# Autodesk Inventor assembly: 2v2 LWL Robot
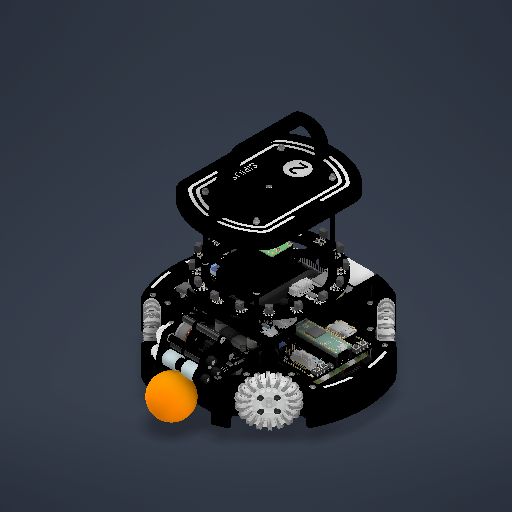
[picture p0: Inventor's stored thumbnail of the model, 512x512]
Saved by Autodesk Inventor 2026.1 (Build 301233020, 233B)
## iProperties
Created: 2026-04-03
Part Number: 2v2 LWL Robot
Document SubType Name: Assembly
Designer: Bahaa
Mass: 1441.25 g
Surface Area: 8202.25 cm^2
Volume: 790.623 cm^3
Density: 1.82292 g/cm^3
Author: Bahaa
## Documents named in this file (23)
- C:\Users\Bahaa\Nextcloud2\CAD\25-26\V2\2v2 LWL Robot.iam
- C:\Users\Bahaa\Nextcloud2\CAD\25-26\V2\Bottom Ring.ipt
- C:\Users\Bahaa\Nextcloud2\CAD\25-26\V2\Motor Assembly.iam
- C:\Users\Bahaa\Nextcloud2\CAD\25-26\V2\Top Ring.ipt
- C:\Users\Bahaa\Nextcloud2\CAD\25-26\V2\Side Wall.ipt
- C:\Users\Bahaa\Nextcloud2\CAD\25-26\V2\Battery Cover.ipt
- C:\Users\Bahaa\Nextcloud2\CAD\25-26\V2\Parts\SLS Quantum 1300mAh 4S1P 14,8V 65C.ipt
- C:\Users\Bahaa\Nextcloud2\CAD\25-26\V2\Solenoid JF-0826B\Solenoid JF-0826B\Solenoid.iam
- C:\Users\Bahaa\Nextcloud2\CAD\25-26\V2\Central Assembly.iam
- C:\Users\Bahaa\Nextcloud2\CAD\25-26\V2\Dribbler\Dribbler V2\Dribbler.iam
- C:\Users\Bahaa\Nextcloud2\CAD\25-26\V2\Ball.ipt
- C:\Users\Bahaa\Documents\Inventor\Content Center Files\R2026\en-US\DIN 7991(2)\DIN 7991 - M3x8.ipt
- C:\Users\Bahaa\Documents\Inventor\Content Center Files\R2026\en-US\DIN 912\DIN 912 - M3 x 0,5 x 5 x 3,75.ipt
- C:\Users\Bahaa\Nextcloud2\CAD\25-26\V2\Boards\Lineboard\Lineboard\Lineboard.iam
- C:\Users\Bahaa\Nextcloud2\CAD\25-26\V2\Boards\Logic Board\Logic Board\Logic Board.iam
- C:\Users\Bahaa\Nextcloud2\CAD\25-26\V2\Boards\Motor Board R\Motor Board R\Motor Board R.iam
- C:\Users\Bahaa\Nextcloud2\CAD\25-26\V2\Boards\Motor Board L\Motor Board L\Motor Board L.iam
- C:\Users\Bahaa\Nextcloud2\CAD\25-26\V2\Boards\Power Board\Power Board\Power Board.iam
- C:\Users\Bahaa\Documents\Inventor\Content Center Files\R2026\en-US\DIN 934\DIN 934 - M3 x 0,5.ipt
- C:\Users\Bahaa\Nextcloud2\CAD\25-26\V2\Boards\Kicker Board\Kicker Board\Kicker Board.iam
- C:\Users\Bahaa\Nextcloud2\CAD\25-26\V2\Parts\LED.ipt
- C:\Users\Bahaa\Nextcloud2\CAD\25-26\V2\Parts\WP3DP3BT.ipt
- C:\Users\Bahaa\Nextcloud2\CAD\25-26\V2\Parts\XL6019 Joy-IT\XL6019 Joy-IT\XL6019 Joy-IT\XL6019 Joy-IT.iam
## Components (44 placed, 22 different names)
1. Central Assembly:1 [sub-assembly] — Mate:53, Mate:54, Mate:55, Insert:1, Insert:2, Insert:3, Insert:4, Insert:5, Insert:6, Insert:7, Insert:8
2. Dribbler:1 [sub-assembly] — Mate:56, Mate:57, Mate:58, Tangent:1, Mate:62, Mate:63
3. Ball:1 — Mate:59, Mate:60, Mate:61
4. Motor Board R:1 [sub-assembly] — Mate:73, Mate:74, Mate:75, Mate:80, Flush:59, Flush:60
5. Motor Board L:1 [sub-assembly] — Mate:76, Mate:77, Mate:78, Mate:79, Flush:57, Flush:58
6. Power Board:1 [sub-assembly] — Mate:80, Flush:59, Flush:60
7. Kicker Board:1 [sub-assembly] — Mate:88, Mate:89, Mate:90, Insert:16, Insert:17
8. LED:1 — Mate:91, Mate:92
9. WP3DP3BT:1 — Mate:93, Mate:94
10. XL6019 Joy-IT:1 [sub-assembly] — Mate:95, Mate:97, Mate:98, Mate:99, Mate:100, Insert:18, Insert:19
11. DIN 934 - replaced by DIN EN 24032/28673/28674 M3:1 — Angle:3, Mate:97
12. DIN 934 - replaced by DIN EN 24032/28673/28674 M3:2 — Mate:96, Angle:4, Mate:98
13. DIN 912 - replaced by DIN EN ISO 4762 M3 x 5:18 — Insert:18
14. DIN 912 - replaced by DIN EN ISO 4762 M3 x 5:19 — Insert:19
15. Bottom Ring:1 — Mate:1, Mate:17, Mate:18, Flush:1, Mate:22, Mate:24, Mate:27, Mate:28, Mate:29, Mate:33, Mate:60, Angle:2, Mate:70, Mate:71, Mate:72, Mate:91, Mate:92, Mate:93, Mate:94
16. Top Ring:1 — Mate:4, Mate:23, Mate:25, Mate:26, Mate:30, Mate:48, Mate:53, Mate:54, Mate:55, Mate:56, Mate:57, Mate:58, Insert:9, Insert:10, Insert:11, Insert:12, Insert:13, Mate:88, Mate:89, Mate:90, Mate:95, Angle:3, Angle:4, Mate:99, Mate:100
17. Lineboard:1 [sub-assembly] — Mate:70, Mate:71, Mate:72
18. Logic Board:1 [sub-assembly] — Mate:79, Flush:57, Flush:58
19. Side Wall:1 — Flush:1, Mate:25, Mate:26, Mate:76, Mate:77, Mate:78
20. Side Wall:2 — Mate:22, Mate:23, Mate:24, Mate:73, Mate:74, Mate:75
21. Battery Cover:1 — Mate:27, Mate:28, Mate:29, Mate:30, Mate:32
22. SLS Quantum 1300mAh 4S1P 14,8V 65C:1 — Mate:32, Mate:33
23. Solenoid:1 [sub-assembly] — Mate:48
24. DIN 912 - replaced by DIN EN ISO 4762 M3 x 5:16 — Insert:16
25. DIN 912 - replaced by DIN EN ISO 4762 M3 x 5:17 — Insert:17
26. DIN 7991 M3x8:1 — Mate:62
27. DIN 7991 M3x8:2 — Mate:63
28. DIN 912 - replaced by DIN EN ISO 4762 M3 x 5:1 — Insert:1
29. DIN 912 - replaced by DIN EN ISO 4762 M3 x 5:2 — Insert:2
30. DIN 912 - replaced by DIN EN ISO 4762 M3 x 5:3 — Insert:3
31. DIN 912 - replaced by DIN EN ISO 4762 M3 x 5:4 — Insert:4
32. DIN 912 - replaced by DIN EN ISO 4762 M3 x 5:5 — Insert:5
33. DIN 912 - replaced by DIN EN ISO 4762 M3 x 5:6 — Insert:6
34. DIN 912 - replaced by DIN EN ISO 4762 M3 x 5:7 — Insert:7
35. DIN 912 - replaced by DIN EN ISO 4762 M3 x 5:8 — Insert:8
36. DIN 912 - replaced by DIN EN ISO 4762 M3 x 5:9 — Insert:9
37. DIN 912 - replaced by DIN EN ISO 4762 M3 x 5:10 — Insert:10
38. DIN 912 - replaced by DIN EN ISO 4762 M3 x 5:11 — Insert:11
39. DIN 912 - replaced by DIN EN ISO 4762 M3 x 5:12 — Insert:12
40. DIN 912 - replaced by DIN EN ISO 4762 M3 x 5:13 — Insert:13
41. Motor Assembly:1 [sub-assembly] — Mate:1, Mate:17, Mate:18
42. Motor Assembly:2 [sub-assembly] — Mate:4
43. Motor Assembly:3 [sub-assembly]
44. Motor Assembly:4 [sub-assembly]
## Component patterns: Motor Assemblies (4 elements)
## Relationships (78: Mate 51, Insert 17, Flush 6, Angle 3, Tangent 1)
- Mate:1: Bottom Ring:1 ↔ Motor Assembly:1
- Mate:4: Top Ring:1 ↔ Motor Assembly:2
- Mate:17: Bottom Ring:1 ↔ Motor Assembly:1
- Mate:18: Bottom Ring:1 ↔ Motor Assembly:1
- Flush:1: Bottom Ring:1 ↔ Side Wall:1
- Mate:22: Bottom Ring:1 ↔ Side Wall:2
- Mate:23: Top Ring:1 ↔ Side Wall:2
- Mate:24: Bottom Ring:1 ↔ Side Wall:2
- Mate:25: Top Ring:1 ↔ Side Wall:1
- Mate:26: Top Ring:1 ↔ Side Wall:1
- Mate:27: Bottom Ring:1 ↔ Battery Cover:1
- Mate:28: Bottom Ring:1 ↔ Battery Cover:1
- Mate:29: Bottom Ring:1 ↔ Battery Cover:1
- Mate:30: Top Ring:1 ↔ Battery Cover:1
- Mate:32 (0.25 mm): Battery Cover:1 ↔ SLS Quantum 1300mAh 4S1P 14,8V 65C:1
- Mate:33 (0.25 mm): Bottom Ring:1 ↔ SLS Quantum 1300mAh 4S1P 14,8V 65C:1
- Mate:48: Top Ring:1 ↔ Solenoid:1
- Mate:53: Central Assembly:1 ↔ Top Ring:1
- Mate:54: Central Assembly:1 ↔ Top Ring:1
- Mate:55: Central Assembly:1 ↔ Top Ring:1
- Mate:56: Dribbler:1 ↔ Top Ring:1
- Mate:57: Dribbler:1 ↔ Top Ring:1
- Mate:58: Dribbler:1 ↔ Top Ring:1
- Flush:56 (-11 mm)
- Mate:59 (21 mm): Ball:1
- Mate:60 (21 mm): Ball:1 ↔ Bottom Ring:1
- Mate:61: Ball:1
- Angle:2 (0 deg): Bottom Ring:1
- Tangent:1: Dribbler:1
- Mate:62: Dribbler:1 ↔ DIN 7991 M3x8:1
- Mate:63: Dribbler:1 ↔ DIN 7991 M3x8:2
- Insert:1: Central Assembly:1 ↔ DIN 912 - replaced by DIN EN ISO 4762 M3 x 5:1
- Insert:2: Central Assembly:1 ↔ DIN 912 - replaced by DIN EN ISO 4762 M3 x 5:2
- Insert:3: Central Assembly:1 ↔ DIN 912 - replaced by DIN EN ISO 4762 M3 x 5:3
- Insert:4: Central Assembly:1 ↔ DIN 912 - replaced by DIN EN ISO 4762 M3 x 5:4
- Insert:5: Central Assembly:1 ↔ DIN 912 - replaced by DIN EN ISO 4762 M3 x 5:5
- Insert:6: Central Assembly:1 ↔ DIN 912 - replaced by DIN EN ISO 4762 M3 x 5:6
- Insert:7: Central Assembly:1 ↔ DIN 912 - replaced by DIN EN ISO 4762 M3 x 5:7
- Insert:8: Central Assembly:1 ↔ DIN 912 - replaced by DIN EN ISO 4762 M3 x 5:8
- Insert:9: Top Ring:1 ↔ DIN 912 - replaced by DIN EN ISO 4762 M3 x 5:9
- Insert:10: Top Ring:1 ↔ DIN 912 - replaced by DIN EN ISO 4762 M3 x 5:10
- Insert:11: Top Ring:1 ↔ DIN 912 - replaced by DIN EN ISO 4762 M3 x 5:11
- Insert:12: Top Ring:1 ↔ DIN 912 - replaced by DIN EN ISO 4762 M3 x 5:12
- Insert:13: Top Ring:1 ↔ DIN 912 - replaced by DIN EN ISO 4762 M3 x 5:13
- Mate:70: Bottom Ring:1 ↔ Lineboard:1
- Mate:71: Bottom Ring:1 ↔ Lineboard:1
- Mate:72: Bottom Ring:1 ↔ Lineboard:1
- Mate:73: Motor Board R:1 ↔ Side Wall:2
- Mate:74: Motor Board R:1 ↔ Side Wall:2
- Mate:75: Motor Board R:1 ↔ Side Wall:2
- Mate:76: Motor Board L:1 ↔ Side Wall:1
- Mate:77: Motor Board L:1 ↔ Side Wall:1
- Mate:78: Motor Board L:1 ↔ Side Wall:1
- Mate:79: Motor Board L:1 ↔ Logic Board:1
- Flush:57: Motor Board L:1 ↔ Logic Board:1
- Flush:58: Motor Board L:1 ↔ Logic Board:1
- Mate:80: Motor Board R:1 ↔ Power Board:1
- Flush:59: Motor Board R:1 ↔ Power Board:1
- Flush:60: Motor Board R:1 ↔ Power Board:1
- Mate:88: Kicker Board:1 ↔ Top Ring:1
- Mate:89: Kicker Board:1 ↔ Top Ring:1
- Mate:90: Kicker Board:1 ↔ Top Ring:1
- Insert:16: Kicker Board:1 ↔ DIN 912 - replaced by DIN EN ISO 4762 M3 x 5:16
- Insert:17: Kicker Board:1 ↔ DIN 912 - replaced by DIN EN ISO 4762 M3 x 5:17
- Mate:91 (3 mm): LED:1 ↔ Bottom Ring:1
- Mate:92: LED:1 ↔ Bottom Ring:1
- Mate:93 (3 mm): WP3DP3BT:1 ↔ Bottom Ring:1
- Mate:94: WP3DP3BT:1 ↔ Bottom Ring:1
- Mate:95: XL6019 Joy-IT:1 ↔ Top Ring:1
- Angle:3 (0 deg): DIN 934 - replaced by DIN EN 24032/28673/28674 M3:1 ↔ Top Ring:1
- Mate:96: DIN 934 - replaced by DIN EN 24032/28673/28674 M3:2
- Angle:4 (0 deg): DIN 934 - replaced by DIN EN 24032/28673/28674 M3:2 ↔ Top Ring:1
- Mate:97: XL6019 Joy-IT:1 ↔ DIN 934 - replaced by DIN EN 24032/28673/28674 M3:1
- Mate:98: XL6019 Joy-IT:1 ↔ DIN 934 - replaced by DIN EN 24032/28673/28674 M3:2
- Mate:99: XL6019 Joy-IT:1 ↔ Top Ring:1
- Mate:100: XL6019 Joy-IT:1 ↔ Top Ring:1
- Insert:18: XL6019 Joy-IT:1 ↔ DIN 912 - replaced by DIN EN ISO 4762 M3 x 5:18
- Insert:19: XL6019 Joy-IT:1 ↔ DIN 912 - replaced by DIN EN ISO 4762 M3 x 5:19
